# Autodesk Inventor assembly: Вентиль
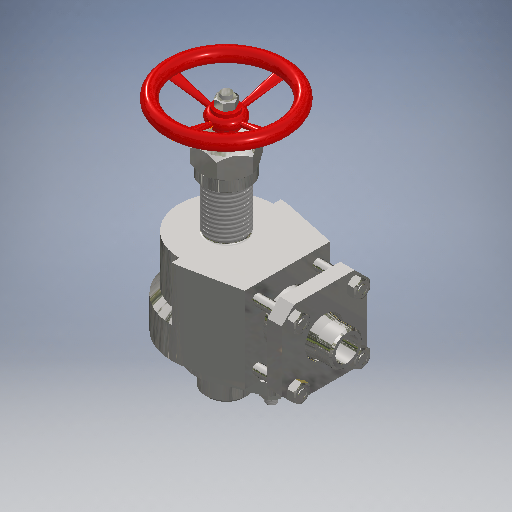
[picture p0: Inventor's stored thumbnail of the model, 512x512]
Saved by Autodesk Inventor 2025.2 (Build 292293000, 293)
## iProperties
Created: 2024-12-20
Part Number: Вентиль
Document SubType Name: Assembly
Designer: Anna
Author: Anna
## Documents named in this file (18)
- E:\inventor\VALVE\VALVE.iam
- E:\inventor\VALVE\00.32.003 Fitting.ipt
- E:\inventor\VALVE\00.32.004 Flange.ipt
- E:\inventor\VALVE\00.32.001 Housing.ipt
- E:\inventor\VALVE\00.32.005 Bushing.ipt
- E:\inventor\VALVE\00.32.002 Fitting.ipt
- E:\inventor\VALVE\00.32.011 Flange.ipt
- E:\inventor\VALVE\00.32.006 Ring.ipt
- E:\inventor\VALVE\00.32.008 Bushing.ipt
- E:\inventor\VALVE\00.32.007 Nut.ipt
- E:\inventor\VALVE\00.32.013 Bushing.ipt
- E:\inventor\VALVE\00.32.012 Valve.ipt
- E:\inventor\VALVE\00.32.010 Spindle.ipt
- E:\inventor\VALVE\00.32.009 Flywheel.ipt
- C:\Users\LOCALADMIN\Documents\Inventor\Content Center Files\R2025\en-US\GOST 5915-70\Nut M12-6H GOST 5915-70.ipt
- E:\inventor\VALVE\M12-6H GOST 5915-70.ipt
- C:\Users\LOCALADMIN\Documents\Inventor\Content Center Files\R2025\en-US\Stud GOST 22034-76\Stud M12-6g×45 GOST 22034-76.ipt
- C:\Users\LOCALADMIN\Documents\Inventor\Content Center Files\R2025\en-US\Stud GOST 22034-76\Stud M12-6g×55 GOST 22034-76.ipt
## Components (26 placed, 17 different names)
1. 00.32.001 Housing:1 — Mate:1, Mate:3, Mate:6, Mate:7, Mate:11, Mate:12, Mate:16, Mate:17, Mate:18, Mate:19
2. 00.32.003 Fitting:1 — Mate:1, Mate:2
3. 00.32.004 Flange:1 — Mate:2, Mate:20, Mate:21, Mate:22, Mate:23
4. 00.32.005 Bushing:1 — Mate:3, Mate:4, Mate:10
5. 00.32.002 Fitting:1 — Mate:4, Mate:5
6. 00.32.011 Flange:1 — Mate:5, Mate:14, Mate:15
7. 00.32.006 Ring:1 — Mate:6
8. 00.32.008 Bushing:1 — Mate:8
9. 00.32.007 Nut:1 — Mate:7, Mate:8
10. 00.32.013 Bushing:1 — Mate:9
11. 00.32.012 Valve:1 — Mate:9, Insert:1, Mate:10
12. 00.32.010 Spindle:1 — Insert:1, Insert:2, Insert:3
13. 00.32.009 Flywheel:1 — Insert:2
14. M12-6H GOST 5915-70:1 — Insert:3
15. Stud GOST 22034-76 M12-6g×45:2 — Mate:11, Mate:13
16. Stud GOST 22034-76 M12-6g×45:3 — Mate:12
17. Nut GOST 5915-70 M12:1 — Mate:13, Mate:15
18. Nut GOST 5915-70 M12:2 — Mate:14
19. Stud GOST 22034-76 M12-6g×55:1 — Mate:17
20. Stud GOST 22034-76 M12-6g×55:2 — Mate:18
21. Stud GOST 22034-76 M12-6g×55:3 — Mate:19
22. Stud GOST 22034-76 M12-6g×55:4 — Mate:16
23. Nut GOST 5915-70 M12:3 — Mate:22
24. Nut GOST 5915-70 M12:4 — Mate:21
25. Nut GOST 5915-70 M12:5 — Mate:23
26. Nut GOST 5915-70 M12:6 — Mate:20
## Relationships (26: Mate 23, Insert 3)
- Mate:1: 00.32.001 Housing:1 ↔ 00.32.003 Fitting:1
- Mate:2: 00.32.003 Fitting:1 ↔ 00.32.004 Flange:1
- Mate:3: 00.32.001 Housing:1 ↔ 00.32.005 Bushing:1
- Mate:4: 00.32.005 Bushing:1 ↔ 00.32.002 Fitting:1
- Mate:5: 00.32.002 Fitting:1 ↔ 00.32.011 Flange:1
- Mate:6: 00.32.001 Housing:1 ↔ 00.32.006 Ring:1
- Mate:7: 00.32.001 Housing:1 ↔ 00.32.007 Nut:1
- Mate:8: 00.32.008 Bushing:1 ↔ 00.32.007 Nut:1
- Mate:9: 00.32.013 Bushing:1 ↔ 00.32.012 Valve:1
- Insert:1 (2.28 mm): 00.32.012 Valve:1 ↔ 00.32.010 Spindle:1
- Mate:10: 00.32.005 Bushing:1 ↔ 00.32.012 Valve:1
- Insert:2: 00.32.010 Spindle:1 ↔ 00.32.009 Flywheel:1
- Insert:3 (4 mm): 00.32.010 Spindle:1 ↔ M12-6H GOST 5915-70:1
- Mate:11: 00.32.001 Housing:1 ↔ Stud GOST 22034-76 M12-6g×45:2
- Mate:12: 00.32.001 Housing:1 ↔ Stud GOST 22034-76 M12-6g×45:3
- Mate:13: Stud GOST 22034-76 M12-6g×45:2 ↔ Nut GOST 5915-70 M12:1
- Mate:14: 00.32.011 Flange:1 ↔ Nut GOST 5915-70 M12:2
- Mate:15: 00.32.011 Flange:1 ↔ Nut GOST 5915-70 M12:1
- Mate:16: 00.32.001 Housing:1 ↔ Stud GOST 22034-76 M12-6g×55:4
- Mate:17: 00.32.001 Housing:1 ↔ Stud GOST 22034-76 M12-6g×55:1
- Mate:18: 00.32.001 Housing:1 ↔ Stud GOST 22034-76 M12-6g×55:2
- Mate:19: 00.32.001 Housing:1 ↔ Stud GOST 22034-76 M12-6g×55:3
- Mate:20: 00.32.004 Flange:1 ↔ Nut GOST 5915-70 M12:6
- Mate:21: 00.32.004 Flange:1 ↔ Nut GOST 5915-70 M12:4
- Mate:22: 00.32.004 Flange:1 ↔ Nut GOST 5915-70 M12:3
- Mate:23: 00.32.004 Flange:1 ↔ Nut GOST 5915-70 M12:5
